# Autodesk Inventor assembly: repisas
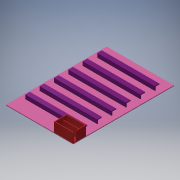
[picture p0: Inventor's stored thumbnail of the model, 180x180]
Saved by Autodesk Inventor 2018 (Build 220112000, 112)
## iProperties
Created: 2018-01-24
Part Number: repisas
Document SubType Name: Assembly
Designer: mokuz
Author: mokuz
## Documents named in this file (4)
- D:\proyectos\pared_agua\repisas.iam
- D:\proyectos\pared_agua\panel.ipt
- D:\proyectos\pared_agua\repisa.ipt
- D:\proyectos\pared_agua\box.ipt
## Components (8 placed, 3 different names)
1. panel:1 — Flush:1, Mate:1, Mate:2, Flush:2, Mate:3, Flush:3
2. box:1 — Flush:2, Mate:3, Flush:3
3. repisa:1 — Flush:1, Mate:1, Mate:2
4. repisa:6
5. repisa:7
6. repisa:8
7. repisa:9
8. repisa:10
## Component patterns: (6 elements, first: repisa:1)
## Relationships (6: Flush 3, Mate 3)
- Flush:1: panel:1 ↔ repisa:1
- Mate:1: panel:1 ↔ repisa:1
- Mate:2: panel:1 ↔ repisa:1
- Flush:2: panel:1 ↔ box:1
- Mate:3: panel:1 ↔ box:1
- Flush:3: panel:1 ↔ box:1
